# Autodesk Inventor assembly: LOZYSKO Z KOSZEM
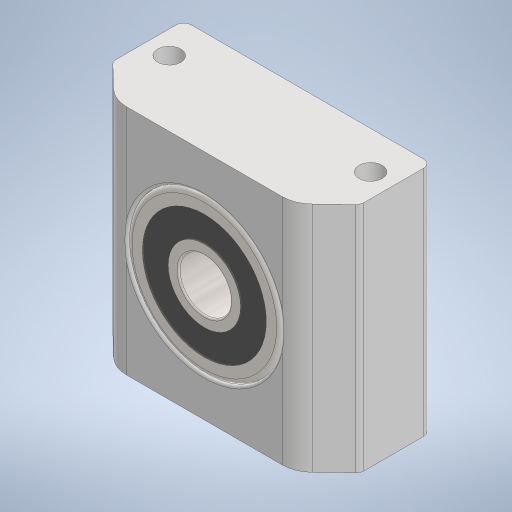
[picture p0: Inventor's stored thumbnail of the model, 512x512]
Saved by Autodesk Inventor 2023 (Build 270158000, 158)
## iProperties
Created: 2023-03-06
Part Number: LOZYSKO Z KOSZEM
Document SubType Name: Assembly
Designer: Kamil
Author: Kamil
## Documents named in this file (3)
- C:\Users\Kamil\Desktop\KONARM\konarm 3 przegub\LOZYSKO Z KOSZEM.iam
- C:\Users\Kamil\Desktop\KONARM\konarm 3 przegub\Uchwyt_na_lozysko_poli.ipt
- C:\Users\Kamil\Downloads\3200_2rs.ipt
## Components (2 placed, 2 different names)
1. Uchwyt_na_lozysko_poli:2 — Zestawiające:1, Zestawiające:2
2. 3200_2rs:1 — Zestawiające:1, Zestawiające:2
## Relationships (2: Mate 2)
- Zestawiające:1 [Mate]: Uchwyt_na_lozysko_poli:2 ↔ 3200_2rs:1
- Zestawiające:2 [Mate]: Uchwyt_na_lozysko_poli:2 ↔ 3200_2rs:1
